# Autodesk Inventor assembly: cnc_assembly_wo_z
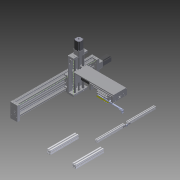
[picture p0: Inventor's stored thumbnail of the model, 180x180]
Saved by Autodesk Inventor 2011 (Build 150239000, 239)
## iProperties
Created: 2012-06-14
Part Number: cnc_assembly_wo_z
Document SubType Name: Assembly
Designer: labuser
Author: labuser
## Documents named in this file (9)
- C:\Users\labuser\Desktop\cnc_cad\cnc_assembly_wo_z.iam
- C:\Users\labuser\Desktop\cnc_cad\New XZ_Combo Master.iam
- C:\Users\labuser\Desktop\cnc_cad\z_axis.iam
- C:\Users\labuser\Desktop\cnc_cad\nema_23.ipt
- C:\Users\labuser\Desktop\cnc_cad\head_assembly.iam
- C:\Users\labuser\Desktop\cnc_cad\l_bracket.ipt
- C:\Users\labuser\Documents\GitHub\kinematic_mount\magnet_chuck_redesign\new_assembly.iam
- C:\Users\labuser\Desktop\cnc_cad\8020-40-4040-Lite.ipt
- C:\Users\labuser\Desktop\cnc_cad\8020-25-2525.ipt
## Components (12 placed, 8 different names)
1. New XZ_Combo Master:1 [sub-assembly] — Mate:1, Mate:3, Mate:11, Mate:12, Mate:13
2. z_axis:1 [sub-assembly] — Mate:5, Mate:6, Mate:7, Mate:8, Mate:9, Mate:10, Mate:14, Mate:15
3. nema_23:1 — Mate:3
4. nema_23:2 — Mate:8, Mate:9, Mate:10
5. nema_23:3 — Mate:1
6. head_assembly:1 [sub-assembly] — Mate:5, Mate:6, Mate:7
7. l_bracket:1 — Mate:11, Mate:12, Mate:13, Mate:14, Mate:15
8. new_assembly:1 [sub-assembly] — Mate:16, Mate:17, Mate:18, Mate:19
9. 8020-40-4040-Lite:1
10. 8020-40-4040-Lite:2
11. 8020-25-2525:1 — Mate:16, Mate:17
12. 8020-25-2525:2 — Mate:18, Mate:19
## Relationships (17: Mate 17)
- Mate:1: New XZ_Combo Master:1 ↔ nema_23:3
- Mate:3: New XZ_Combo Master:1 ↔ nema_23:1
- Mate:5: z_axis:1 ↔ head_assembly:1
- Mate:6: z_axis:1 ↔ head_assembly:1
- Mate:7: z_axis:1 ↔ head_assembly:1
- Mate:8: z_axis:1 ↔ nema_23:2
- Mate:9: z_axis:1 ↔ nema_23:2
- Mate:10: z_axis:1 ↔ nema_23:2
- Mate:11: New XZ_Combo Master:1 ↔ l_bracket:1
- Mate:12: New XZ_Combo Master:1 ↔ l_bracket:1
- Mate:13: New XZ_Combo Master:1 ↔ l_bracket:1
- Mate:14: z_axis:1 ↔ l_bracket:1
- Mate:15: z_axis:1 ↔ l_bracket:1
- Mate:16: new_assembly:1 ↔ 8020-25-2525:1
- Mate:17: new_assembly:1 ↔ 8020-25-2525:1
- Mate:18: new_assembly:1 ↔ 8020-25-2525:2
- Mate:19: new_assembly:1 ↔ 8020-25-2525:2
